# Autodesk Inventor assembly: XY-Axis Connection
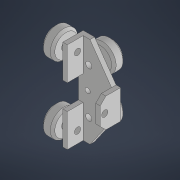
[picture p0: Inventor's stored thumbnail of the model, 180x180]
Saved by Autodesk Inventor 2022 (Build 260153000, 153)
## iProperties
Created: 2023-06-15
Part Number: XY-Axis Connection
Document SubType Name: Assembly
Designer: Ryan Mitcham
Author: Ryan Mitcham
## Documents named in this file (3)
- C:\Users\Gaming\OneDrive\Documents\Inventor\XYZ-Gantry\XY-Axis Connection\XY-Axis Connection.iam
- C:\Users\Gaming\OneDrive\Documents\Inventor\XYZ-Gantry\XY-Axis Connection\Wheel Mount.ipt
- C:\Users\Gaming\OneDrive\Documents\Inventor\XYZ-Gantry\Standard Parts\20x20 Extrusion Compatible Wheel.ipt
## Components (5 placed, 2 different names)
1. Wheel Mount:1 — Mate:1, Mate:2, Mate:3, Mate:4, Mate:5, Mate:6, Mate:7, Mate:8, Mate:9, Mate:10, Mate:11
2. 20x20 Extrusion Compatible Wheel:1 — Mate:6, Mate:7
3. 20x20 Extrusion Compatible Wheel:2 — Mate:8, Mate:9
4. 20x20 Extrusion Compatible Wheel:3 — Mate:10, Mate:11
5. 20x20 Extrusion Compatible Wheel:4 — Mate:4, Mate:5
## Relationships (11: Mate 11)
- Mate:1: Wheel Mount:1
- Mate:2: Wheel Mount:1
- Mate:3: Wheel Mount:1
- Mate:4: Wheel Mount:1 ↔ 20x20 Extrusion Compatible Wheel:4
- Mate:5: Wheel Mount:1 ↔ 20x20 Extrusion Compatible Wheel:4
- Mate:6: Wheel Mount:1 ↔ 20x20 Extrusion Compatible Wheel:1
- Mate:7: Wheel Mount:1 ↔ 20x20 Extrusion Compatible Wheel:1
- Mate:8: Wheel Mount:1 ↔ 20x20 Extrusion Compatible Wheel:2
- Mate:9: Wheel Mount:1 ↔ 20x20 Extrusion Compatible Wheel:2
- Mate:10: Wheel Mount:1 ↔ 20x20 Extrusion Compatible Wheel:3
- Mate:11: Wheel Mount:1 ↔ 20x20 Extrusion Compatible Wheel:3
